# Autodesk Inventor assembly: Drukpers
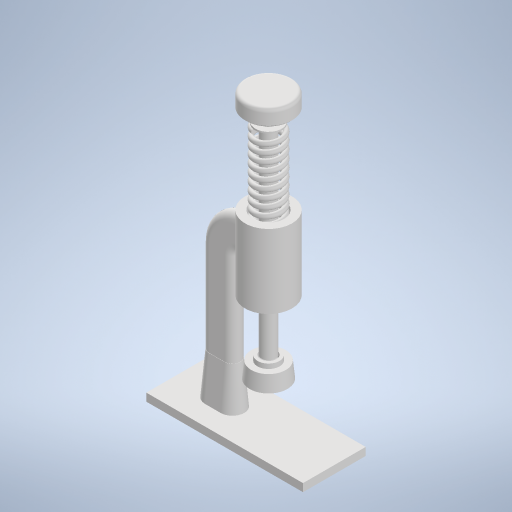
[picture p0: Inventor's stored thumbnail of the model, 512x512]
Saved by Autodesk Inventor 2023 (Build 270158000, 158)
## iProperties
Created: 2022-11-18
Part Number: Drukpers
Document SubType Name: Assembly
Designer: Ayoub
Author: Ayoub
## Documents named in this file (6)
- C:\Users\Ayoub\Documents\GitHub\zonnepaneel-concept\Parts\Drukpers.iam
- C:\Users\Ayoub\Documents\GitHub\School\Inventor\School\drukpers.ipt
- C:\Users\Ayoub\Documents\GitHub\School\Inventor\School\as.ipt
- C:\Users\Ayoub\Documents\GitHub\School\Inventor\School\handvat.ipt
- C:\Users\Ayoub\Documents\GitHub\School\Inventor\School\perskop.ipt
- C:\Users\Ayoub\Documents\GitHub\School\Inventor\School\veer.ipt
## Components (5 placed, 5 different names)
1. drukpers:1 — Mate:1, Mate:2, Mate:3, Flush:1
2. as:1 — Mate:3, Mate:4, Mate:5, Mate:6, Mate:7
3. handvat:1 — Mate:4, Mate:6
4. perskop:1 — Mate:5, Mate:7, Mate:8
5. veer:1 — Mate:1, Mate:2
## Relationships (9: Mate 8, Flush 1)
- Mate:1: drukpers:1 ↔ veer:1
- Mate:2: drukpers:1 ↔ veer:1
- Mate:3: drukpers:1 ↔ as:1
- Mate:4: as:1 ↔ handvat:1
- Mate:5: as:1 ↔ perskop:1
- Mate:6: as:1 ↔ handvat:1
- Mate:7: as:1 ↔ perskop:1
- Flush:1 (27 mm): drukpers:1
- Mate:8: perskop:1
